# Autodesk Inventor assembly: ロボットベース
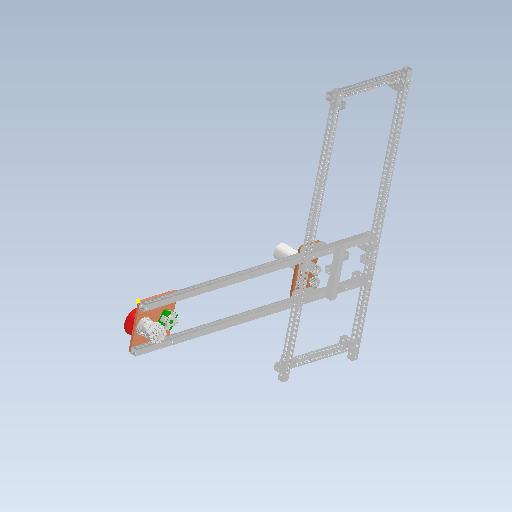
[picture p0: Inventor's stored thumbnail of the model, 512x512]
Saved by Autodesk Inventor 2020.3 (Build 243373000, 373)
## iProperties
Created: 2020-07-04
Part Number: ロボットベース
Document SubType Name: Assembly
Designer: totot
Mass: 1046.74 g
Surface Area: 4640.27 cm^2
Volume: 552.45 cm^3
Density: 1.89472 g/cm^3
Author: totot
## Documents named in this file (15)
- D:\mysvn\ロボコン\キャチロボ\キャチロボ設計図\ロボット\ロボットベース\ロボットベース.iam
- D:\mysvn\ロボコン\キャチロボ\キャチロボ設計図\ロボット\ロボットベース\ロボットベース15x15_1.ipt
- D:\mysvn\ロボコン\キャチロボ\キャチロボ設計図\ロボット\ロボットベース\ロボットベース15x15_2.ipt
- D:\mysvn\ロボコン\キャチロボ\キャチロボ設計図\ロボット\ロボットベース\ロボットベース15x15x30.ipt
- D:\mysvn\ロボコン\キャチロボ\キャチロボ設計図\ロボット\ロボットベース\ロボットベース15x15x15.ipt
- D:\mysvn\ロボコン\キャチロボ\キャチロボ設計図\ロボット\ロボットベース\ロボットベース15x15_3.ipt
- D:\mysvn\ロボコン\キャチロボ\キャチロボ設計図\ロボット\ロボットベース\ロボットベース15x15_4.ipt
- D:\mysvn\ロボコン\キャチロボ\キャチロボ設計図\ロボット\ロボットベース\ロボットベース15x15_5.ipt
- D:\mysvn\ロボコン\キャチロボ\キャチロボ設計図\ロボット\ロボットベース\ロボットベースT5.5.ipt
- D:\mysvn\ロボコン\キャチロボ\キャチロボ設計図\ロボット\共有パーツ\RS_540.ipt
- D:\mysvn\ロボコン\キャチロボ\キャチロボ設計図\ロボット\共有パーツ\PS1-20_On.ipt
- D:\mysvn\ロボコン\キャチロボ\キャチロボ設計図\ロボット\共有パーツ\ポテンションメーター_BI-7284.ipt
- D:\mysvn\ロボコン\キャチロボ\キャチロボ設計図\ロボット\共有パーツ\cad_STEP_OUTSIDE-APN1nnDN.iam
- D:\mysvn\ロボコン\キャチロボ\キャチロボ設計図\ロボット\共有パーツ\cad_STEP_OUTSIDE-XN1E-BV5##M.iam
- D:\mysvn\ロボコン\キャチロボ\キャチロボ設計図\ロボットベースT5.5_2.ipt
## Components (29 placed, 14 different names)
1. ロボットベース15x15_1:2 — 挿入:2, 挿入:3, 挿入:11, 挿入:13, 挿入:20, 挿入:23, 挿入:40, 挿入:57
2. ロボットベース15x15_1:1 — 挿入:4, 挿入:6, 挿入:8, 挿入:10, 挿入:12, 挿入:34, 挿入:37, 挿入:38, 挿入:42
3. ロボットベース15x15_2:1 — 挿入:38, 挿入:39, 挿入:40, 挿入:41
4. ロボットベース15x15x30:1 — 挿入:39, 挿入:42
5. ロボットベース15x15x30:2 — 挿入:23, 挿入:41
6. ロボットベース15x15x30:3 — 挿入:1, 挿入:3
7. ロボットベース15x15x30:4 — 挿入:5, 挿入:6
8. ロボットベース15x15_2:2 — 挿入:1, 挿入:2, 挿入:4, 挿入:5
9. ロボットベース15x15_3:1 — 挿入:10, 挿入:11, 挿入:21, 挿入:25, 挿入:26, 挿入:27, 挿入:35, 挿入:45, 挿入:51, 挿入:52
10. ロボットベース15x15x15:1 — 挿入:8
11. ロボットベース15x15x30:6 — 挿入:43, 挿入:44
12. ロボットベース15x15_3:2 — 挿入:12, 挿入:13, 挿入:24, 挿入:28, 挿入:29, 挿入:36, 挿入:43, 挿入:53, 挿入:54, 挿入:56
13. ロボットベース15x15x15:2 — 挿入:49
14. ロボットベース15x15x30:7 — 挿入:34, 挿入:35
15. ロボットベース15x15x30:8 — 挿入:36, 挿入:37
16. ロボットベース15x15_4:1 — 挿入:24, 挿入:25, 挿入:44, 挿入:47, 挿入:49
17. ロボットベース15x15x30:9 — 挿入:20, 挿入:21
18. ロボットベース15x15x30:10 — 挿入:45, 挿入:47
19. ロボットベース15x15_5:1 — 挿入:26, 挿入:27, 挿入:30, 挿入:31, 挿入:32
20. ロボットベース15x15_5:2 — 挿入:28, 挿入:29, 挿入:33
21. ロボットベースT5.5:1 — 挿入:17, 挿入:18, 挿入:19, 挿入:30, 挿入:31, 挿入:32, 挿入:33, 挿入:46
22. RS_540:1 — 挿入:17, 挿入:18, 挿入:19, 挿入:22
23. PS1-20_On:1 — 挿入:22
24. ポテンションメーター_BI-7284:1 — 挿入:46, 挿入:48
25. PS1-20_On:2 — 挿入:48
26. cad_STEP_OUTSIDE-APN1nnDN:1 [sub-assembly] — 挿入:55
27. cad_STEP_OUTSIDE-XN1E-BV5##M:1 [sub-assembly] — 挿入:50
28. ロボットベースT5.5_2:1 — 挿入:50, 挿入:51, 挿入:52, 挿入:53, 挿入:54, 挿入:55
29. ロボットベース15x15x30:11 — 挿入:56, 挿入:57
## Relationships (52: Insert 52)
- 挿入:1 [Insert]: ロボットベース15x15x30:3 ↔ ロボットベース15x15_2:2
- 挿入:2 [Insert]: ロボットベース15x15_1:2 ↔ ロボットベース15x15_2:2
- 挿入:3 [Insert]: ロボットベース15x15_1:2 ↔ ロボットベース15x15x30:3
- 挿入:4 [Insert]: ロボットベース15x15_1:1 ↔ ロボットベース15x15_2:2
- 挿入:5 [Insert]: ロボットベース15x15x30:4 ↔ ロボットベース15x15_2:2
- 挿入:6 [Insert]: ロボットベース15x15_1:1 ↔ ロボットベース15x15x30:4
- 挿入:8 [Insert]: ロボットベース15x15_1:1 ↔ ロボットベース15x15x15:1
- 挿入:10 [Insert]: ロボットベース15x15_1:1 ↔ ロボットベース15x15_3:1
- 挿入:11 [Insert]: ロボットベース15x15_1:2 ↔ ロボットベース15x15_3:1
- 挿入:12 [Insert]: ロボットベース15x15_1:1 ↔ ロボットベース15x15_3:2
- 挿入:13 [Insert]: ロボットベース15x15_1:2 ↔ ロボットベース15x15_3:2
- 挿入:17 [Insert]: ロボットベースT5.5:1 ↔ RS_540:1
- 挿入:18 [Insert]: ロボットベースT5.5:1 ↔ RS_540:1
- 挿入:19 [Insert]: ロボットベースT5.5:1 ↔ RS_540:1
- 挿入:20 [Insert]: ロボットベース15x15_1:2 ↔ ロボットベース15x15x30:9
- 挿入:21 [Insert]: ロボットベース15x15_3:1 ↔ ロボットベース15x15x30:9
- 挿入:22 [Insert]: RS_540:1 ↔ PS1-20_On:1
- 挿入:23 [Insert]: ロボットベース15x15_1:2 ↔ ロボットベース15x15x30:2
- 挿入:24 [Insert]: ロボットベース15x15_3:2 ↔ ロボットベース15x15_4:1
- 挿入:25 [Insert]: ロボットベース15x15_3:1 ↔ ロボットベース15x15_4:1
- 挿入:26 [Insert]: ロボットベース15x15_3:1 ↔ ロボットベース15x15_5:1
- 挿入:27 [Insert]: ロボットベース15x15_3:1 ↔ ロボットベース15x15_5:1
- 挿入:28 [Insert]: ロボットベース15x15_3:2 ↔ ロボットベース15x15_5:2
- 挿入:29 [Insert]: ロボットベース15x15_3:2 ↔ ロボットベース15x15_5:2
- 挿入:30 [Insert]: ロボットベース15x15_5:1 ↔ ロボットベースT5.5:1
- 挿入:31 [Insert]: ロボットベース15x15_5:1 ↔ ロボットベースT5.5:1
- 挿入:32 [Insert]: ロボットベース15x15_5:1 ↔ ロボットベースT5.5:1
- 挿入:33 [Insert]: ロボットベース15x15_5:2 ↔ ロボットベースT5.5:1
- 挿入:34 [Insert]: ロボットベース15x15_1:1 ↔ ロボットベース15x15x30:7
- 挿入:35 [Insert]: ロボットベース15x15_3:1 ↔ ロボットベース15x15x30:7
- 挿入:36 [Insert]: ロボットベース15x15_3:2 ↔ ロボットベース15x15x30:8
- 挿入:37 [Insert]: ロボットベース15x15_1:1 ↔ ロボットベース15x15x30:8
- 挿入:38 [Insert]: ロボットベース15x15_1:1 ↔ ロボットベース15x15_2:1
- 挿入:39 [Insert]: ロボットベース15x15_2:1 ↔ ロボットベース15x15x30:1
- 挿入:40 [Insert]: ロボットベース15x15_1:2 ↔ ロボットベース15x15_2:1
- 挿入:41 [Insert]: ロボットベース15x15_2:1 ↔ ロボットベース15x15x30:2
- 挿入:42 [Insert]: ロボットベース15x15_1:1 ↔ ロボットベース15x15x30:1
- 挿入:43 [Insert]: ロボットベース15x15x30:6 ↔ ロボットベース15x15_3:2
- 挿入:44 [Insert]: ロボットベース15x15x30:6 ↔ ロボットベース15x15_4:1
- 挿入:45 [Insert]: ロボットベース15x15_3:1 ↔ ロボットベース15x15x30:10
- 挿入:46 [Insert]: ロボットベースT5.5:1 ↔ ポテンションメーター_BI-7284:1
- 挿入:47 [Insert]: ロボットベース15x15_4:1 ↔ ロボットベース15x15x30:10
- 挿入:48 [Insert]: ポテンションメーター_BI-7284:1 ↔ PS1-20_On:2
- 挿入:49 [Insert]: ロボットベース15x15x15:2 ↔ ロボットベース15x15_4:1
- 挿入:50 [Insert]: cad_STEP_OUTSIDE-XN1E-BV5##M:1 ↔ ロボットベースT5.5_2:1
- 挿入:51 [Insert]: ロボットベース15x15_3:1 ↔ ロボットベースT5.5_2:1
- 挿入:52 [Insert]: ロボットベース15x15_3:1 ↔ ロボットベースT5.5_2:1
- 挿入:53 [Insert]: ロボットベース15x15_3:2 ↔ ロボットベースT5.5_2:1
- 挿入:54 [Insert]: ロボットベース15x15_3:2 ↔ ロボットベースT5.5_2:1
- 挿入:55 [Insert]: cad_STEP_OUTSIDE-APN1nnDN:1 ↔ ロボットベースT5.5_2:1
- 挿入:56 [Insert]: ロボットベース15x15_3:2 ↔ ロボットベース15x15x30:11
- 挿入:57 [Insert]: ロボットベース15x15_1:2 ↔ ロボットベース15x15x30:11
